# Autodesk Inventor assembly: STEFAN
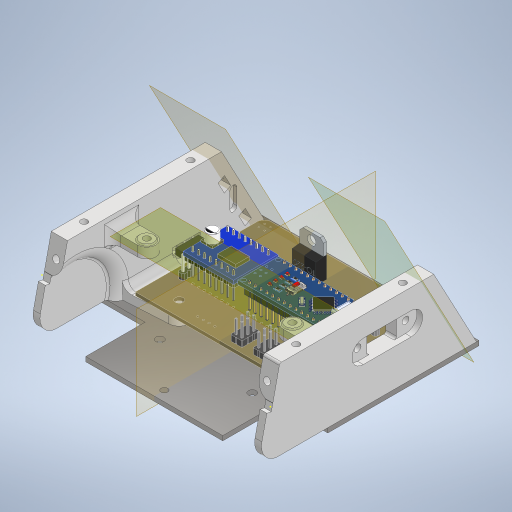
[picture p0: Inventor's stored thumbnail of the model, 512x512]
Saved by Autodesk Inventor 2023 (Build 270158000, 158)
## iProperties
Created: 2023-07-07
Part Number: STEFAN
Document SubType Name: Assembly
Designer: Kamil
Author: Kamil
## Documents named in this file (24)
- C:\Users\Kamil\Desktop\MojeRoboty\Stefan\mechanics 2\STEFAN.iam
- C:\Users\Kamil\Desktop\MojeRoboty\Stefan\mechanics 2\podstawa.ipt
- C:\Users\Kamil\Desktop\MojeRoboty\Stefan\mechanics 2\n20 motor.ipt
- C:\Users\Kamil\Desktop\MojeRoboty\Stefan\mechanics 2\plytka_dol.iam
- C:\Users\Kamil\Desktop\MojeRoboty\Stefan\mechanics 2\GP2Y0A41SK0F.ipt
- C:\Users\Kamil\Desktop\MojeRoboty\Stefan\mechanics 2\dach.ipt
- C:\Users\Kamil\Desktop\MojeRoboty\Stefan\mechanics 2\servo_mini_1370hd_cos.ipt
- C:\Users\Kamil\Desktop\MojeRoboty\Stefan\mechanics 2\oko.ipt
- C:\Users\Kamil\Desktop\MojeRoboty\Stefan\mechanics 2\buzia.ipt
- C:\Users\Kamil\Desktop\MojeRoboty\Stefan\mechanics 2\reka.ipt
- C:\Users\Kamil\Desktop\MojeRoboty\Stefan\mechanics 2\board_up.ipt
- C:\Users\Kamil\Desktop\MojeRoboty\Stefan\mechanics 2\plug_2.ipt
- C:\Users\Kamil\Desktop\MojeRoboty\Stefan\mechanics 2\zaslepka.ipt
- C:\Users\Kamil\Desktop\MojeRoboty\Stefan\mechanics 2\uchwyt_silnikow.ipt
- C:\Users\Kamil\Desktop\MojeRoboty\Stefan\mechanics 2\uchwyt_serw.ipt
- C:\Users\Kamil\Desktop\sciana_awaryjna.ipt
- C:\Users\Kamil\Desktop\MojeRoboty\Stefan\mechanics 2\kolo.ipt
- C:\Users\Kamil\Desktop\MojeRoboty\Stefan\mechanics 2\opona.ipt
- C:\Users\Kamil\Desktop\MojeRoboty\Stefan\mechanics 2\tylna.ipt
- C:\Users\Kamil\Desktop\MojeRoboty\Stefan\mechanics 2\mocowanie sharpow.ipt
- C:\Users\Kamil\Desktop\MojeRoboty\Stefan\mechanics 2\szkic.ipt
- C:\Users\Kamil\Desktop\MojeRoboty\Stefan\mechanics 2\plug_kopia.ipt
- C:\Users\Kamil\Desktop\MojeRoboty\Stefan\mechanics 2\SCIANA_LEWA_NOWA_2.ipt
- C:\Users\Kamil\Desktop\MojeRoboty\Stefan\mechanics 2\wlacznik_2.ipt
## Components (29 placed, 23 different names)
1. podstawa:1 — Równoległe:4, Równoległe:10, Równoległe:14, Równoległe:21, Zestawiające:39, Zestawiające:40, Zestawiające:41, Zestawiające:45, Zestawiające:46, Zestawiające:58, Symetria:1, Zestawiające:65, Zestawiające:66
2. n20 motor:1 — Równoległe:4, Zestawiające:51, Zestawiające:54
3. n20 motor:2 — Zestawiające:52, Zestawiające:53
4. plytka_dol:1 [sub-assembly] — Równoległe:19, Zestawiające:47, Zestawiające:58, Zestawiające:59, Zestawiające:61, Równoległe:31
5. GP2Y0A41SK0F:1 — Zestawiające:62, Zestawiające:63, Zestawiające:64
6. dach:1 — Równoległe:10, Zestawiające:24, Zestawiające:25, Równoległe:13, Zestawiające:42, Zestawiające:55, Zestawiające:56
7. servo_mini_1370hd_cos:1 — Zestawiające:25, Zestawiające:26, Równoległe:12, Równoległe:13, Zestawiające:35, Zestawiające:36, Zestawiające:43, Zestawiające:44
8. servo_mini_1370hd_cos:2 — Zestawiające:24, Zestawiające:26, Równoległe:12, Równoległe:14, Zestawiające:37, Zestawiające:38
9. oko:1
10. oko:2
11. buzia:1
12. reka:1 — Zestawiające:35, Zestawiające:36
13. reka:2 — Zestawiające:37, Zestawiające:38
14. board_up:1 — Równoległe:19, Zestawiające:48
15. plug_2:1 — Równoległe:21, Równoległe:27, Równoległe:28, Równoległe:29
16. zaslepka:1
17. uchwyt_silnikow:1 — Zestawiające:39, Zestawiające:40, Zestawiające:41
18. uchwyt_serw:1 — Zestawiające:42, Zestawiające:43, Zestawiające:44, Zestawiające:55, Zestawiające:56
19. sciana_awaryjna:1 — Zestawiające:45, Zestawiające:46, Zestawiające:47, Zestawiające:48, Równoległe:24, Zestawiające:59, Symetria:1, Równoległe:26, Równoległe:30
20. kolo:1 — Zestawiające:49, Zestawiające:51, Zestawiające:54, Równoległe:22
21. kolo:2 — Zestawiające:50, Zestawiające:52, Zestawiające:53, Równoległe:23
22. opona:1 — Zestawiające:49, Równoległe:23, Równoległe:25
23. opona:2 — Zestawiające:50, Równoległe:22
24. tylna:1 — Równoległe:24
25. mocowanie sharpow:1 — Zestawiające:60, Równoległe:26, Zestawiające:61, Zestawiające:62, Zestawiające:63, Zestawiające:64
26. szkic:1 — Równoległe:25
27. plug_kopia:1 — Równoległe:27, Równoległe:28, Równoległe:29
28. SCIANA_LEWA_NOWA_2:1 — Zestawiające:65, Równoległe:30, Zestawiające:66
29. wlacznik_2:1 — Równoległe:31
## Relationships (52: Mate 34, Flush 17, Symmetry 1)
- Równoległe:4 [Flush]: podstawa:1 ↔ n20 motor:1
- Równoległe:10 [Flush]: podstawa:1 ↔ dach:1
- Zestawiające:24 [Mate]: dach:1 ↔ servo_mini_1370hd_cos:2
- Zestawiające:25 [Mate]: dach:1 ↔ servo_mini_1370hd_cos:1
- Zestawiające:26 [Mate] (5 mm): servo_mini_1370hd_cos:1 ↔ servo_mini_1370hd_cos:2
- Równoległe:12 [Flush]: servo_mini_1370hd_cos:1 ↔ servo_mini_1370hd_cos:2
- Równoległe:13 [Flush] (10 mm): dach:1 ↔ servo_mini_1370hd_cos:1
- Równoległe:14 [Flush] (27.5 mm): podstawa:1 ↔ servo_mini_1370hd_cos:2
- Zestawiające:35 [Mate] (1 mm): servo_mini_1370hd_cos:1 ↔ reka:1
- Zestawiające:36 [Mate]: servo_mini_1370hd_cos:1 ↔ reka:1
- Zestawiające:37 [Mate] (1 mm): servo_mini_1370hd_cos:2 ↔ reka:2
- Zestawiające:38 [Mate]: servo_mini_1370hd_cos:2 ↔ reka:2
- Równoległe:19 [Flush]: plytka_dol:1 ↔ board_up:1
- Równoległe:21 [Flush]: podstawa:1 ↔ plug_2:1
- Zestawiające:39 [Mate]: podstawa:1 ↔ uchwyt_silnikow:1
- Zestawiające:40 [Mate]: podstawa:1 ↔ uchwyt_silnikow:1
- Zestawiające:41 [Mate]: podstawa:1 ↔ uchwyt_silnikow:1
- Zestawiające:42 [Mate]: dach:1 ↔ uchwyt_serw:1
- Zestawiające:43 [Mate]: servo_mini_1370hd_cos:1 ↔ uchwyt_serw:1
- Zestawiające:44 [Mate]: servo_mini_1370hd_cos:1 ↔ uchwyt_serw:1
- Zestawiające:45 [Mate]: podstawa:1 ↔ sciana_awaryjna:1
- Zestawiające:46 [Mate]: podstawa:1 ↔ sciana_awaryjna:1
- Zestawiające:47 [Mate]: plytka_dol:1 ↔ sciana_awaryjna:1
- Zestawiające:48 [Mate]: board_up:1 ↔ sciana_awaryjna:1
- Zestawiające:49 [Mate]: kolo:1 ↔ opona:1
- Zestawiające:50 [Mate]: kolo:2 ↔ opona:2
- Zestawiające:51 [Mate]: n20 motor:1 ↔ kolo:1
- Zestawiające:52 [Mate]: n20 motor:2 ↔ kolo:2
- Zestawiające:53 [Mate]: n20 motor:2 ↔ kolo:2
- Zestawiające:54 [Mate]: n20 motor:1 ↔ kolo:1
- Równoległe:22 [Flush]: kolo:1 ↔ opona:2
- Równoległe:23 [Flush]: kolo:2 ↔ opona:1
- Równoległe:24 [Flush]: sciana_awaryjna:1 ↔ tylna:1
- Zestawiające:55 [Mate]: dach:1 ↔ uchwyt_serw:1
- Zestawiające:56 [Mate]: dach:1 ↔ uchwyt_serw:1
- Równoległe:25 [Flush]: opona:1 ↔ szkic:1
- Zestawiające:58 [Mate]: podstawa:1 ↔ plytka_dol:1
- Zestawiające:59 [Mate]: plytka_dol:1 ↔ sciana_awaryjna:1
- Symetria:1 [Symmetry]: podstawa:1 ↔ sciana_awaryjna:1
- Zestawiające:60 [Mate]: mocowanie sharpow:1
- Równoległe:26 [Flush]: sciana_awaryjna:1 ↔ mocowanie sharpow:1
- Zestawiające:61 [Mate] (2 mm): plytka_dol:1 ↔ mocowanie sharpow:1
- Zestawiające:62 [Mate]: GP2Y0A41SK0F:1 ↔ mocowanie sharpow:1
- Zestawiające:63 [Mate]: GP2Y0A41SK0F:1 ↔ mocowanie sharpow:1
- Zestawiające:64 [Mate]: GP2Y0A41SK0F:1 ↔ mocowanie sharpow:1
- Równoległe:27 [Flush]: plug_2:1 ↔ plug_kopia:1
- Równoległe:28 [Flush]: plug_2:1 ↔ plug_kopia:1
- Równoległe:29 [Flush]: plug_2:1 ↔ plug_kopia:1
- Zestawiające:65 [Mate]: podstawa:1 ↔ SCIANA_LEWA_NOWA_2:1
- Równoległe:30 [Flush]: sciana_awaryjna:1 ↔ SCIANA_LEWA_NOWA_2:1
- Zestawiające:66 [Mate]: podstawa:1 ↔ SCIANA_LEWA_NOWA_2:1
- Równoległe:31 [Flush]: plytka_dol:1 ↔ wlacznik_2:1
